# Autodesk Inventor assembly: Assembly1
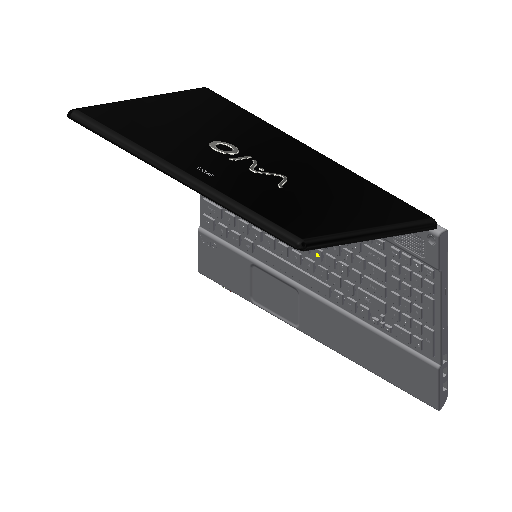
[picture p0: Inventor's stored thumbnail of the model, 512x512]
Saved by Autodesk Inventor 2022 (Build 260153000, 153)
## iProperties
Created: 2017-08-02
Part Number: Assembly1
Document SubType Name: Assembly
Designer: avik
Author: avik
## Documents named in this file (3)
- C:\Users\ferna\Downloads\sony-vaio-laptop-2.snapshot.4\Assembly1.iam
- C:\Users\ferna\Downloads\sony-vaio-laptop-2.snapshot.4\KEYBOARD.ipt
- C:\Users\ferna\Downloads\sony-vaio-laptop-2.snapshot.4\LED.ipt
## Components (2 placed, 2 different names)
1. KEYBOARD:1 — Mate:1, Mate:2
2. LED:1 — Mate:1, Mate:2
## Relationships (2: Mate 2)
- Mate:1: KEYBOARD:1 ↔ LED:1
- Mate:2 (0.5 mm): KEYBOARD:1 ↔ LED:1
